# Autodesk Inventor assembly: 2nd LawAssembly
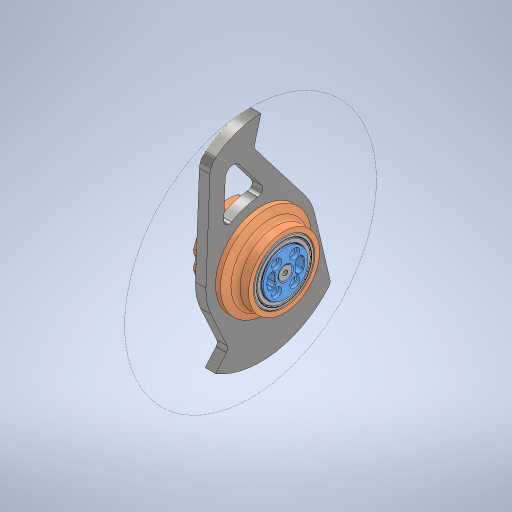
[picture p0: Inventor's stored thumbnail of the model, 512x512]
Saved by Autodesk Inventor 2023.4 (Build 274418000, 418)
## iProperties
Created: 2024-05-28
Part Number: 2nd LawAssembly
Document SubType Name: Assembly
Designer: Nathan Cai
Mass: 419.962 g
Surface Area: 579.686 cm^2
Volume: 75.8127 cm^3
Density: 5.53947 g/cm^3
Author: Nathan Cai
## Documents named in this file (3)
- E:\Documents\Inventor\Law - V2.1\2nd Law\2nd Law Assembly.iam
- E:\Documents\Inventor\Law - V2.1\2nd Law\Battle Ready Motor RDY 5536 V1.2 v12 PRODUCTION\Battle Ready Motor RDY 5536 V1.2 v12 PRODUCTION.iam
- E:\Documents\Inventor\Law - V2.1\2nd Law\Blade.ipt
## Components (2 placed, 2 different names)
1. Battle Ready Motor RDY 5536 V1.2 v12 PRODUCTION:1 [sub-assembly] — Mate:1, Mate:2, Mate:3
2. Blade:1 — Mate:1, Mate:2, Mate:3
## Relationships (3: Mate 3)
- Mate:1: Battle Ready Motor RDY 5536 V1.2 v12 PRODUCTION:1 ↔ Blade:1
- Mate:2: Battle Ready Motor RDY 5536 V1.2 v12 PRODUCTION:1 ↔ Blade:1
- Mate:3: Battle Ready Motor RDY 5536 V1.2 v12 PRODUCTION:1 ↔ Blade:1
